# Autodesk Inventor assembly: back_plates
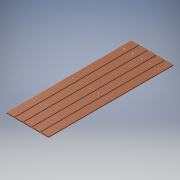
[picture p0: Inventor's stored thumbnail of the model, 180x180]
Saved by Autodesk Inventor 2019 (Build 230136000, 136)
## iProperties
Created: 2019-02-23
Part Number: back_plates
Document SubType Name: Assembly
Designer: gaincarlo
Author: gaincarlo
## Documents named in this file (4)
- D:\Giancarlo Bacchio\Documenti\00 - Progetti\30-Inventor\LaPanca-Baraca\back_plates.iam
- D:\Giancarlo Bacchio\Documenti\00 - Progetti\30-Inventor\LaPanca-Baraca\support1.ipt
- D:\Giancarlo Bacchio\Documenti\00 - Progetti\30-Inventor\LaPanca-Baraca\doga_long1.ipt
- D:\Giancarlo Bacchio\Documenti\Inventor\Content Center Files\R2019\en-US\GB_T 15-88\Bolt GB_T 15 M8 x 35.ipt
## Components (23 placed, 3 different names)
1. support1:1 — Mate:1, Mate:2, Mate:7
2. support1:2 — Mate:3, Mate:5, Mate:9
3. support1:3 — Mate:4, Mate:6, Mate:8
4. doga_long1:1 — Mate:1, Mate:2, Mate:3, Mate:4, Mate:5, Mate:6
5. doga_long1:2
6. doga_long1:3 — Mate:7, Mate:8, Mate:9
7. doga_long1:4 — Mate:10, Mate:11
8. doga_long1:5
9. Bolt GB/T 15-1988 M8x35:1 — Mate:10, Mate:11
10. Bolt GB/T 15-1988 M8x35:2
11. Bolt GB/T 15-1988 M8x35:3
12. Bolt GB/T 15-1988 M8x35:4
13. Bolt GB/T 15-1988 M8x35:5
14. Bolt GB/T 15-1988 M8x35:6
15. Bolt GB/T 15-1988 M8x35:7
16. Bolt GB/T 15-1988 M8x35:8
17. Bolt GB/T 15-1988 M8x35:9
18. Bolt GB/T 15-1988 M8x35:10
19. Bolt GB/T 15-1988 M8x35:11
20. Bolt GB/T 15-1988 M8x35:12
21. Bolt GB/T 15-1988 M8x35:13
22. Bolt GB/T 15-1988 M8x35:14
23. Bolt GB/T 15-1988 M8x35:15
## Component patterns: (5 elements, first: doga_long1:1), (15 elements, first: Bolt GB/T 15-1988 M8x35:1)
## Relationships (11: Mate 11)
- Mate:1: support1:1 ↔ doga_long1:1
- Mate:2: support1:1 ↔ doga_long1:1
- Mate:3: support1:2 ↔ doga_long1:1
- Mate:4: support1:3 ↔ doga_long1:1
- Mate:5: support1:2 ↔ doga_long1:1
- Mate:6: support1:3 ↔ doga_long1:1
- Mate:7: support1:1 ↔ doga_long1:3
- Mate:8: support1:3 ↔ doga_long1:3
- Mate:9: support1:2 ↔ doga_long1:3
- Mate:10: doga_long1:4 ↔ Bolt GB/T 15-1988 M8x35:1
- Mate:11: doga_long1:4 ↔ Bolt GB/T 15-1988 M8x35:1
